# Autodesk Inventor assembly: Assembly3
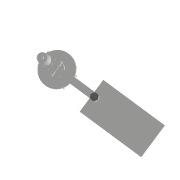
[picture p0: Inventor's stored thumbnail of the model, 180x180]
Saved by Autodesk Inventor 2022 (Build 260153000, 153)
## iProperties
Created: 2021-07-24
Part Number: Assembly3
Document SubType Name: Assembly
Designer: LENOVO
Author: LENOVO
## Documents named in this file (7)
- C:\Users\LENOVO\Documents\Inventor\explo\Assembly3.iam
- C:\Users\LENOVO\Documents\Inventor\explo\Uptop2.ipt
- C:\Users\LENOVO\Documents\Inventor\explo\FINAL_MOP.iam
- C:\Users\LENOVO\Documents\Inventor\explo\BOLT-HH-A193-B8M-316\BOLT-HH-A193-SS-0.75-3.00.ipt
- C:\Users\LENOVO\Documents\Inventor\explo\BOLT-HH-A193-B8M-316.ipt
- C:\Users\LENOVO\Documents\Inventor\explo\NUT-HEX-A194 8M-SS\NUT-HEX-A194-8M-SS-0.750.ipt
- C:\Users\LENOVO\Documents\Inventor\explo\NUT-HEX-A194 8M-SS.ipt
## Components (4 placed, 4 different names)
1. Uptop2:1 — Rigid:1, Rigid:2
2. FINAL_MOP:1 [sub-assembly] — Rotational:1, Rigid:1
3. BOLT-HH-A193-SS-0.75-3.00:1 — Rotational:1
4. NUT-HEX-A194-8M-SS-0.750:1 — Rigid:2
## Relationships (3: WeldJoint 2, RevoluteJoint 1)
- Rotational:1 [RevoluteJoint]: FINAL_MOP:1 ↔ BOLT-HH-A193-SS-0.75-3.00:1
- Rigid:1 [WeldJoint]: Uptop2:1 ↔ FINAL_MOP:1
- Rigid:2 [WeldJoint]: Uptop2:1 ↔ NUT-HEX-A194-8M-SS-0.750:1
